# Autodesk Inventor assembly: Wasp Pivot Shaft
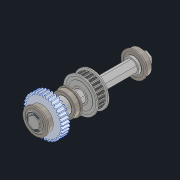
[picture p0: Inventor's stored thumbnail of the model, 180x180]
Saved by Autodesk Inventor 2022 (Build 260153000, 153)
## iProperties
Created: 2022-09-18
Part Number: Wasp Pivot Shaft
Document SubType Name: Assembly
Designer: robpl
Author: robpl
## Documents named in this file (9)
- C:\Users\robpl\OneDrive\Documents\Inventor\WASP\Wasp\Wasp Pivot Shaft.iam
- C:\Users\robpl\OneDrive\Documents\Inventor\WASP\Wasp\Wasp Pivot Axle.ipt
- C:\Users\robpl\OneDrive\Documents\Inventor\WASP\Wasp\0.5 Flanged Hex Bearing (1.125 OD) (217-3875).ipt
- C:\Users\robpl\OneDrive\Documents\Inventor\WASP\Wasp\36T Aluminum Spur Gear (20 DP, 1_2_ Hex Bore) (217-3214).ipt
- C:\Users\robpl\OneDrive\Documents\Inventor\WASP\Wasp\24T x 9mm Wide Double Flange Aluminum Pulley (HTD 5mm, 1_2” Hex Bore) (217-3227) (1).ipt
- C:\Users\robpl\OneDrive\Documents\Inventor\WASP\Wasp\14.5mm 0.5in Hex Spacer.ipt
- C:\Users\robpl\OneDrive\Documents\Inventor\WASP\Wasp\10mm E-Clip.ipt
- C:\Users\robpl\OneDrive\Documents\Inventor\WASP\Wasp\1mm 0.5in Hex Spacer.ipt
- C:\Users\robpl\OneDrive\Documents\Inventor\WASP\Wasp\2mm 0.5in Hex Spacer.ipt
## Components (12 placed, 8 different names)
1. Wasp Pivot Axle:1 — Mate:1, Mate:2, Flush:1, Mate:3, Mate:4, Mate:6, Mate:7, Mate:17, Mate:18, Mate:25, Mate:26, Mate:27, Mate:28, Angle:1
2. 0.5 Flanged Hex Bearing (1.125 OD) (217-3875):1 — Mate:3, Mate:4, Mate:5, Mate:15, Mate:21, Mate:24, Mate:32, Mate:41
3. 0.5 Flanged Hex Bearing (1.125 OD) (217-3875):2 — Mate:1, Mate:2, Flush:1, Mate:5, Mate:20
4. 36T Aluminum Spur Gear (20 DP, 1_2_ Hex Bore) (217-3214):1 — Mate:6, Mate:7, Mate:20, Mate:22
5. 0.5 Flanged Hex Bearing (1.125 OD) (217-3875):3 — Mate:15, Mate:24, Angle:1, Mate:43, Mate:44
6. 24T x 9mm Wide Double Flange Aluminum Pulley (HTD 5mm, 1_2” Hex Bore) (217-3227) (1):1 — Mate:17, Mate:18, Mate:31
7. 14.5mm 0.5in Hex Spacer:1 — Mate:21, Mate:22
8. 10mm E-Clip:1 — Mate:27, Mate:28, Mate:40
9. 10mm E-Clip:2 — Mate:25, Mate:26
10. 1mm 0.5in Hex Spacer:2 — Mate:31, Mate:32, Mate:42
11. 1mm 0.5in Hex Spacer:3 — Mate:40, Mate:41, Mate:42
12. 2mm 0.5in Hex Spacer:1 — Mate:43, Mate:44
## Relationships (27: Mate 25, Flush 1, Angle 1)
- Mate:1: Wasp Pivot Axle:1 ↔ 0.5 Flanged Hex Bearing (1.125 OD) (217-3875):2
- Mate:2: Wasp Pivot Axle:1 ↔ 0.5 Flanged Hex Bearing (1.125 OD) (217-3875):2
- Flush:1: Wasp Pivot Axle:1 ↔ 0.5 Flanged Hex Bearing (1.125 OD) (217-3875):2
- Mate:3: Wasp Pivot Axle:1 ↔ 0.5 Flanged Hex Bearing (1.125 OD) (217-3875):1
- Mate:4: Wasp Pivot Axle:1 ↔ 0.5 Flanged Hex Bearing (1.125 OD) (217-3875):1
- Mate:5 (40 mm): 0.5 Flanged Hex Bearing (1.125 OD) (217-3875):1 ↔ 0.5 Flanged Hex Bearing (1.125 OD) (217-3875):2
- Mate:6: Wasp Pivot Axle:1 ↔ 36T Aluminum Spur Gear (20 DP, 1_2_ Hex Bore) (217-3214):1
- Mate:7: Wasp Pivot Axle:1 ↔ 36T Aluminum Spur Gear (20 DP, 1_2_ Hex Bore) (217-3214):1
- Mate:15: 0.5 Flanged Hex Bearing (1.125 OD) (217-3875):1 ↔ 0.5 Flanged Hex Bearing (1.125 OD) (217-3875):3
- Mate:17: Wasp Pivot Axle:1 ↔ 24T x 9mm Wide Double Flange Aluminum Pulley (HTD 5mm, 1_2” Hex Bore) (217-3227) (1):1
- Mate:18: Wasp Pivot Axle:1 ↔ 24T x 9mm Wide Double Flange Aluminum Pulley (HTD 5mm, 1_2” Hex Bore) (217-3227) (1):1
- Mate:20: 0.5 Flanged Hex Bearing (1.125 OD) (217-3875):2 ↔ 36T Aluminum Spur Gear (20 DP, 1_2_ Hex Bore) (217-3214):1
- Mate:21: 0.5 Flanged Hex Bearing (1.125 OD) (217-3875):1 ↔ 14.5mm 0.5in Hex Spacer:1
- Mate:22: 36T Aluminum Spur Gear (20 DP, 1_2_ Hex Bore) (217-3214):1 ↔ 14.5mm 0.5in Hex Spacer:1
- Mate:24 (-80 mm): 0.5 Flanged Hex Bearing (1.125 OD) (217-3875):1 ↔ 0.5 Flanged Hex Bearing (1.125 OD) (217-3875):3
- Mate:25: Wasp Pivot Axle:1 ↔ 10mm E-Clip:2
- Mate:26: Wasp Pivot Axle:1 ↔ 10mm E-Clip:2
- Mate:27: Wasp Pivot Axle:1 ↔ 10mm E-Clip:1
- Mate:28: Wasp Pivot Axle:1 ↔ 10mm E-Clip:1
- Mate:31: 24T x 9mm Wide Double Flange Aluminum Pulley (HTD 5mm, 1_2” Hex Bore) (217-3227) (1):1 ↔ 1mm 0.5in Hex Spacer:2
- Mate:32: 0.5 Flanged Hex Bearing (1.125 OD) (217-3875):1 ↔ 1mm 0.5in Hex Spacer:2
- Angle:1 (0 deg): Wasp Pivot Axle:1 ↔ 0.5 Flanged Hex Bearing (1.125 OD) (217-3875):3
- Mate:40: 10mm E-Clip:1 ↔ 1mm 0.5in Hex Spacer:3
- Mate:41: 0.5 Flanged Hex Bearing (1.125 OD) (217-3875):1 ↔ 1mm 0.5in Hex Spacer:3
- Mate:42 (8.3 mm): 1mm 0.5in Hex Spacer:2 ↔ 1mm 0.5in Hex Spacer:3
- Mate:43: 0.5 Flanged Hex Bearing (1.125 OD) (217-3875):3 ↔ 2mm 0.5in Hex Spacer:1
- Mate:44: 0.5 Flanged Hex Bearing (1.125 OD) (217-3875):3 ↔ 2mm 0.5in Hex Spacer:1
